# Autodesk Inventor assembly: LaptopTopDisplay
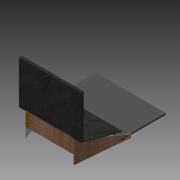
[picture p0: Inventor's stored thumbnail of the model, 180x180]
Saved by Autodesk Inventor 2017 (Build 210142000, 142)
## iProperties
Created: 2018-10-12
Part Number: LaptopTopDisplay
Document SubType Name: Assembly
Designer: ari
Author: ari
## Documents named in this file (7)
- C:\Users\ari\Documents\Inventor\LaptopTopDisplay\LaptopTopDisplay.iam
- C:\Users\ari\Documents\Inventor\LaptopTopDisplay\laptop.ipt
- C:\Users\ari\Documents\Inventor\LaptopTopDisplay\extDisplay.ipt
- C:\Users\ari\Documents\Inventor\LaptopTopDisplay\Stand.ipt
- C:\Users\ari\Documents\Inventor\LaptopTopDisplay\Stand_MIR.ipt
- C:\Users\ari\Documents\Inventor\LaptopTopDisplay\stand_bottom.ipt
- C:\Users\ari\Documents\Inventor\LaptopTopDisplay\scharnierband.ipt
## Components (7 placed, 6 different names)
1. laptop:1 — Mate:2, Mate:3, Angle:1, Flush:3
2. extDisplay:1 — Mate:2, Mate:3, Angle:1, Flush:1, Mate:4, Mate:7, Mate:8, Mate:14
3. Stand:1 — Mate:4, Mate:5, Mate:13, Mate:15
4. Stand_MIR:1 — Mate:6, Mate:7, Mate:8, Mate:10, Mate:14
5. stand_bottom:1 — Mate:5, Flush:3, Mate:6, Mate:9, Mate:12, Flush:6, Flush:7, Mate:15
6. scharnierband:1 — Mate:9, Mate:10, Flush:7
7. scharnierband:2 — Mate:12, Mate:13, Flush:6
## Relationships (18: Mate 13, Flush 4, Angle 1)
- Mate:2 (5 mm): laptop:1 ↔ extDisplay:1
- Mate:3 (-25 mm): laptop:1 ↔ extDisplay:1
- Angle:1 (165 deg): laptop:1 ↔ extDisplay:1
- Flush:1: extDisplay:1
- Mate:4 (0.5 mm): extDisplay:1 ↔ Stand:1
- Mate:5 (0.5 mm): Stand:1 ↔ stand_bottom:1
- Flush:3: laptop:1 ↔ stand_bottom:1
- Mate:6 (0.5 mm): Stand_MIR:1 ↔ stand_bottom:1
- Mate:7 (0.5 mm): extDisplay:1 ↔ Stand_MIR:1
- Mate:8 (0.5 mm): extDisplay:1 ↔ Stand_MIR:1
- Mate:9: stand_bottom:1 ↔ scharnierband:1
- Mate:10: Stand_MIR:1 ↔ scharnierband:1
- Mate:12: stand_bottom:1 ↔ scharnierband:2
- Mate:13: Stand:1 ↔ scharnierband:2
- Flush:6: stand_bottom:1 ↔ scharnierband:2
- Mate:14 (0.5 mm): extDisplay:1 ↔ Stand_MIR:1
- Flush:7: stand_bottom:1 ↔ scharnierband:1
- Mate:15: Stand:1 ↔ stand_bottom:1
